# Autodesk Inventor assembly: Assembly1
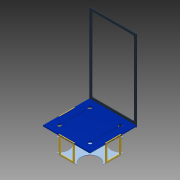
[picture p0: Inventor's stored thumbnail of the model, 180x180]
Saved by Autodesk Inventor 2011 (Build 150239000, 239)
## iProperties
Created: 2011-08-21
Part Number: Assembly1
Document SubType Name: Assembly
Designer: Matthew
Author: Matthew
## Documents named in this file (6)
- C:\Users\Matthew\Documents\matthew_autocad\prlite\base\Assembly1.iam
- C:\Users\Matthew\Documents\matthew_autocad\prlite\base\back.ipt
- C:\Users\Matthew\Documents\matthew_autocad\prlite\base\base top.ipt
- C:\Users\Matthew\Documents\matthew_autocad\prlite\base\base top2.ipt
- C:\Users\Matthew\Documents\matthew_autocad\prlite\base\base bottom.ipt
- C:\Users\Matthew\Documents\matthew_autocad\prlite\base\top-bot connector.ipt
## Components (7 placed, 5 different names)
1. back:1 — Mate:1, Mate:2, Flush:1, Flush:2, Mate:4, Flush:3, Flush:4, Mate:5
2. base top:1 — Mate:1, Mate:2, Flush:1, Mate:3, Mate:8, Flush:5, Mate:11
3. base top2:1 — Mate:3, Flush:2, Mate:4, Flush:6, Mate:10
4. base bottom:1 — Flush:3, Flush:4, Mate:5, Mate:6, Mate:7, Mate:9, Flush:7
5. top-bot connector:1 — Mate:10, Flush:7, Mate:11
6. top-bot connector:2 — Mate:6, Mate:7, Mate:8
7. top-bot connector:3 — Flush:5, Flush:6, Mate:9
## Relationships (18: Mate 11, Flush 7)
- Mate:1: back:1 ↔ base top:1
- Mate:2: back:1 ↔ base top:1
- Flush:1: back:1 ↔ base top:1
- Mate:3: base top:1 ↔ base top2:1
- Flush:2: back:1 ↔ base top2:1
- Mate:4: back:1 ↔ base top2:1
- Flush:3: back:1 ↔ base bottom:1
- Flush:4: back:1 ↔ base bottom:1
- Mate:5: back:1 ↔ base bottom:1
- Mate:6: base bottom:1 ↔ top-bot connector:2
- Mate:7: base bottom:1 ↔ top-bot connector:2
- Mate:8: base top:1 ↔ top-bot connector:2
- Flush:5: base top:1 ↔ top-bot connector:3
- Flush:6: base top2:1 ↔ top-bot connector:3
- Mate:9: base bottom:1 ↔ top-bot connector:3
- Mate:10: base top2:1 ↔ top-bot connector:1
- Flush:7: base bottom:1 ↔ top-bot connector:1
- Mate:11: base top:1 ↔ top-bot connector:1
